# Autodesk Inventor assembly: Ball Shifter shifting 110mm shaft with gears
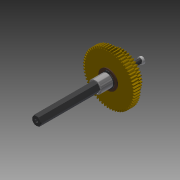
[picture p0: Inventor's stored thumbnail of the model, 180x180]
Saved by Autodesk Inventor 2013 (Build 170138000, 138)
## iProperties
Created: 2013-04-08
Part Number: Ball Shifter shifting 110mm shaft with gears
Document SubType Name: Assembly
Designer: Niemitalo_Dan
Author: Niemitalo_Dan
## Documents named in this file (6)
- \\lmss\students\Robotics\CAD Files\COTS Parts\Gearboxes\Components\VexPro Ball Shifters\Ball Shifter shifting 110mm shaft with gears.iam
- \\lmss\students\Robotics\CAD Files\COTS Parts\Gearboxes\Components\VexPro Ball Shifters\Ballshifter shaft washer.ipt
- \\lmss\students\Robotics\CAD Files\COTS Parts\Gears - VexPro\Gear 20dp ball shifter 60T Vex.ipt
- \\lmss\students\Robotics\CAD Files\COTS Parts\Gears - VexPro\Gear 20dp ball shifter 44T Vex.ipt
- \\lmss\students\Robotics\CAD Files\COTS Parts\Gearboxes\Components\VexPro Ball Shifters\Snap Ring for 750 shaft.ipt
- \\lmss\students\Robotics\CAD Files\COTS Parts\Gearboxes\Components\VexPro Ball Shifters\Ball Shifter 110mm Shaft assy.iam
## Components (5 placed, 5 different names)
1. Ball Shifter 110mm Shaft assy:1 [sub-assembly] — Insert:1, Insert:4
2. Ballshifter shaft washer:1 — Insert:1, Insert:2
3. Gear 20dp ball shifter 60T Vex:1 — Insert:3
4. Gear 20dp ball shifter 44T Vex:1 — Insert:2, Insert:3
5. Snap Ring for 750 shaft:1 — Insert:4
## Relationships (4: Insert 4)
- Insert:1: Ball Shifter 110mm Shaft assy:1 ↔ Ballshifter shaft washer:1
- Insert:2: Ballshifter shaft washer:1 ↔ Gear 20dp ball shifter 44T Vex:1
- Insert:3: Gear 20dp ball shifter 60T Vex:1 ↔ Gear 20dp ball shifter 44T Vex:1
- Insert:4: Ball Shifter 110mm Shaft assy:1 ↔ Snap Ring for 750 shaft:1
